# Autodesk Inventor assembly: Tape Measure Scaler Assembly
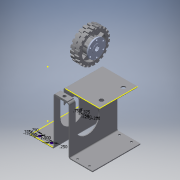
[picture p0: Inventor's stored thumbnail of the model, 180x180]
Saved by Autodesk Inventor 2016 (Build 200138000, 138)
## iProperties
Created: 2016-02-03
Part Number: Tape Measure Scaler Assembly
Document SubType Name: Assembly
Designer: GEH-Magnet School 1
Author: GEH-Magnet School 1
## Documents named in this file (5)
- C:\Users\Andrew\Documents\GitHub\2016RobotCADFiles\Scaler\Tape Measure Scaler Assembly.iam
- C:\Users\Andrew\Documents\GitHub\2016RobotCADFiles\Scaler\Tape Measure Dispenser Part 2.ipt
- C:\Users\Andrew\Documents\GitHub\2016RobotCADFiles\Scaler\Tape Measure Dispenser Side 1.ipt
- C:\Users\Andrew\Documents\GitHub\2016RobotCADFiles\Shooter\4 in HiGrip Wheel.ipt
- C:\Users\Andrew\Documents\GitHub\2016RobotCADFiles\Shooter\am-0096a+500+Hex+Hub+r2.ipt
## Components (4 placed, 4 different names)
1. Tape Measure Dispenser Part 2:1 — Flush:1, Mate:1, Mate:2
2. Tape Measure Dispenser Side 1:1 — Flush:1, Mate:1, Mate:2
3. 4 in HiGrip Wheel:1 — Mate:3, Mate:4, Mate:5
4. am-0096a+500+Hex+Hub+r2:1 — Mate:3, Mate:4, Mate:5
## Relationships (6: Mate 5, Flush 1)
- Flush:1: Tape Measure Dispenser Part 2:1 ↔ Tape Measure Dispenser Side 1:1
- Mate:1: Tape Measure Dispenser Part 2:1 ↔ Tape Measure Dispenser Side 1:1
- Mate:2 (3.302 mm): Tape Measure Dispenser Part 2:1 ↔ Tape Measure Dispenser Side 1:1
- Mate:3: 4 in HiGrip Wheel:1 ↔ am-0096a+500+Hex+Hub+r2:1
- Mate:4: 4 in HiGrip Wheel:1 ↔ am-0096a+500+Hex+Hub+r2:1
- Mate:5: 4 in HiGrip Wheel:1 ↔ am-0096a+500+Hex+Hub+r2:1
